# Autodesk Inventor assembly: eye_bearing
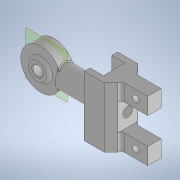
[picture p0: Inventor's stored thumbnail of the model, 180x180]
Saved by Autodesk Inventor 2020 (Build 240168000, 168)
## iProperties
Created: 2020-01-21
Part Number: eye_bearing
Document SubType Name: Assembly
Designer: psrobotics
Author: psrobotics
## Documents named in this file (4)
- F:\projects-3\delta arm\hardware\eye_bearing.iam
- F:\projects-3\delta arm\hardware\eye_bearing_2.ipt
- F:\projects-3\delta arm\hardware\eye_bearing_1.ipt
- F:\projects-3\delta arm\hardware\bbearing_holder_1.ipt
## Components (3 placed, 3 different names)
1. eye_bearing_2:1 — Tangent:1, Flush:1, Insert:1, Angle:2
2. eye_bearing_1:1 — Tangent:1
3. bbearing_holder_1:1 — Flush:1, Insert:1, Angle:2
## Relationships (4: Tangent 1, Flush 1, Insert 1, Angle 1)
- Tangent:1: eye_bearing_2:1 ↔ eye_bearing_1:1
- Flush:1: eye_bearing_2:1 ↔ bbearing_holder_1:1
- Insert:1: eye_bearing_2:1 ↔ bbearing_holder_1:1
- Angle:2 (0 deg): eye_bearing_2:1 ↔ bbearing_holder_1:1
